# Autodesk Inventor assembly: CombinedPiHolder
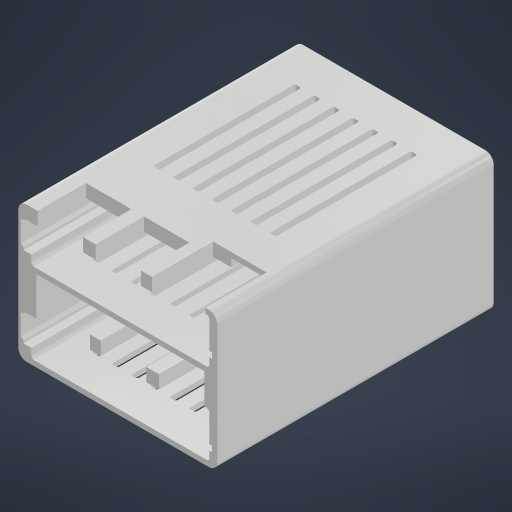
[picture p0: Inventor's stored thumbnail of the model, 512x512]
Saved by Autodesk Inventor 2023 (Build 270158000, 158)
## iProperties
Created: 2023-02-13
Part Number: CombinedPiHolder
Document SubType Name: Assembly
Designer: uzair
Author: uzair
## Documents named in this file (3)
- C:\Users\uzair\Programming\Capstone-MJ02\documentation\3D Models\CombinedPiHolder.iam
- C:\Users\uzair\Programming\Capstone-MJ02\documentation\3D Models\Raspberry_Pi_4_Sleeve_v1-0_MAIN.ipt
- C:\Users\uzair\Programming\Capstone-MJ02\documentation\3D Models\Raspberry_Pi_B+_Sleeve_v2-1_MAIN.ipt
## Components (2 placed, 2 different names)
1. Raspberry_Pi_4_Sleeve_v1-0_MAIN:1 — Mate:1, Mate:2
2. Raspberry_Pi_B+_Sleeve_v2-1_MAIN:1 — Mate:1, Mate:2
## Relationships (2: Mate 2)
- Mate:1: Raspberry_Pi_4_Sleeve_v1-0_MAIN:1 ↔ Raspberry_Pi_B+_Sleeve_v2-1_MAIN:1
- Mate:2: Raspberry_Pi_4_Sleeve_v1-0_MAIN:1 ↔ Raspberry_Pi_B+_Sleeve_v2-1_MAIN:1
